# Autodesk Inventor assembly: Motor
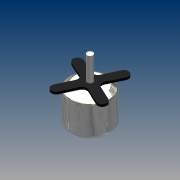
[picture p0: Inventor's stored thumbnail of the model, 180x180]
Saved by Autodesk Inventor 2011 SP1 (Build 150282100, 282)
## iProperties
Created: 2011-07-19
Part Number: Motor
Document SubType Name: Assembly
Designer: Nathan
Author: Nathan
## Documents named in this file (3)
- C:\Users\Nathan\Documents\Inventor\Quadcopter\Motor.iam
- C:\Users\Nathan\Documents\Inventor\Quadcopter\MotorTop.ipt
- C:\Users\Nathan\Documents\Inventor\Quadcopter\MotorBottom.ipt
## Components (2 placed, 2 different names)
1. MotorTop:1 — Mate:1, Mate:2
2. MotorBottom:1 — Mate:1, Mate:2
## Relationships (2: Mate 2)
- Mate:1: MotorTop:1 ↔ MotorBottom:1
- Mate:2: MotorTop:1 ↔ MotorBottom:1
